# Autodesk Inventor assembly: Hand ASM
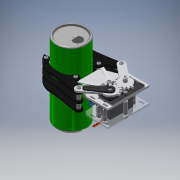
[picture p0: Inventor's stored thumbnail of the model, 180x180]
Saved by Autodesk Inventor 2016 (Build 200138000, 138)
## iProperties
Created: 2017-03-27
Part Number: Hand ASM
Document SubType Name: Assembly
Designer: Nanjar
Author: Nanjar
## Documents named in this file (20)
- D:\Autodesk Invertor prj\Hand Tino Prj2\Hand ASM - Grip.iam
- D:\Autodesk Invertor prj\tower-pro-mg-995-analog-servo-1.snapshot.5\TOWER PRO MG-995, ANALOG SERVO.iam
- D:\Autodesk Invertor prj\Hand Tino Prj\ser Horn.ipt
- D:\Autodesk Invertor prj\Hand Tino Prj\gearb2a.ipt
- D:\Autodesk Invertor prj\Hand Tino Prj\arm1b.ipt
- D:\Autodesk Invertor prj\Hand Tino Prj\claw2.ipt
- D:\Autodesk Invertor prj\Hand Tino Prj\gearb2b.ipt
- D:\Autodesk Invertor prj\arm\spacer 6mm.ipt
- D:\Autodesk Invertor prj\arm\spacer 10mm.ipt
- D:\Autodesk Invertor prj\Gear\Nut90591A121.ipt
- D:\Autodesk Invertor prj\Hand Tino Prj2\Dock bot2.ipt
- D:\Autodesk Invertor prj\Gear\14Screw92005A124.ipt
- D:\Autodesk Invertor prj\Gear\LNut90576A102.ipt
- D:\Autodesk Invertor prj\Gear\10Screw92005A120.ipt
- D:\Autodesk Invertor prj\Gear\20Screw92005A128.ipt
- D:\Autodesk Invertor prj\Hand Tino Prj2\Dock bot1 V2.ipt
- D:\Autodesk Invertor prj\arm\spacer 19mm.ipt
- D:\Autodesk Invertor prj\Downloaded\User Library-HC-SR04\User Library-HC-SR04.iam
- D:\Autodesk Invertor prj\Hand Tino Prj2\Dock top2 V2.ipt
- D:\Autodesk Invertor prj\Hand Tino Prj2\Can1.ipt
## Components (75 placed, 19 different names)
1. TOWER PRO MG-995, ANALOG SERVO:1 [sub-assembly] — Mate:1, Mate:2, Mate:7, Mate:80, Mate:112, Mate:113, Mate:171, Mate:172, Mate:173, Mate:174, Mate:177, Mate:178, Mate:179, Mate:180, Mate:183, Mate:184, Mate:185, Mate:186, Mate:193, Mate:194, Mate:196
2. ser Horn:1 — Mate:1, Mate:2, Mate:6, Mate:8, Mate:81
3. gearb2a:1 — Mate:6, Mate:7, Mate:8, Flush:1, Mate:13, Flush:2, Mate:14, Mate:15, Mate:17, Mate:31, Mate:60, Mate:63, Mate:64, Angle:1, Mate:93, Mate:94, Rotation:1
4. arm1b:1 — Mate:30, Mate:33, Mate:35, Mate:44, Mate:48, Mate:51, Mate:54, Mate:57, Mate:107
5. arm1b:2 — Mate:12, Mate:32, Mate:36, Mate:37, Mate:45, Mate:53, Mate:59, Mate:62, Mate:66
6. claw2:1 — Mate:29, Mate:30, Mate:33, Mate:34, Mate:40, Mate:41, Mate:99, Mate:100, Mate:287, Mate:288, Mate:290
7. claw2:2 — Mate:12, Mate:31, Mate:32, Mate:38, Mate:39, Mate:97, Mate:98, Mate:291, Mate:292, Mate:293, Mate:294
8. gearb2b:1 — Flush:1, Mate:16, Mate:17, Mate:29, Mate:47, Mate:50, Mate:56, Mate:69, Mate:72, Mate:79, Mate:95, Mate:96, Rotation:1
9. spacer 10mm:2 — Mate:34, Mate:35, Mate:49
10. spacer 10mm:3 — Mate:36, Mate:37, Mate:61
11. spacer 10mm:4 — Mate:38, Mate:39
12. spacer 10mm:5 — Mate:40, Mate:41
13. Dock bot2:1 — Mate:44, Mate:45, Mate:51, Mate:53, Mate:107, Mate:110, Mate:111, Mate:299, Mate:300, Mate:301
14. claw2:3 — Mate:47, Mate:48, Mate:49, Mate:52, Mate:55, Mate:313
15. spacer 10mm:7 — Mate:54, Mate:55, Mate:58, Mate:267
16. spacer 10mm:8 — Mate:50, Mate:52, Mate:266
17. claw2:4 — Mate:56, Mate:57, Mate:58, Mate:262, Mate:264, Mate:316
18. claw2:5 — Mate:59, Mate:60, Mate:61, Mate:65, Mate:67, Mate:311
19. claw2:6 — Mate:62, Mate:63, Mate:68, Mate:263, Mate:265, Mate:314
20. spacer 10mm:9 — Mate:64, Mate:65, Mate:268
21. spacer 10mm:10 — Mate:66, Mate:67, Mate:68, Mate:269
22. 14Screw92005A124:1 — Mate:72, Mate:77, Mate:309
23. Nut90591A121:2 — Mate:69, Mate:78, Mate:79
24. LNut90576A102:1 — Mate:77, Mate:78
25. 10Screw92005A120:1 — Mate:80, Mate:81
26. Nut90591A121:3
27. 10Screw92005A120:5 — Mate:93, Mate:94
28. 10Screw92005A120:7 — Mate:95, Mate:96
29. 10Screw92005A120:8 — Mate:97, Mate:98
30. 10Screw92005A120:9 — Mate:99, Mate:100
31. 20Screw92005A128:1 — Mate:283, Mate:305, Mate:308
32. 20Screw92005A128:2 — Mate:110
33. 20Screw92005A128:3 — Mate:111, Mate:270
34. Dock bot1 V2:1 — Mate:112, Mate:113, Mate:189, Mate:190, Mate:191, Mate:192, Mate:197, Mate:198, Mate:199, Mate:200, Mate:271, Mate:272, Mate:273, Mate:274, Mate:276, Mate:278, Mate:280, Mate:282, Mate:284, Mate:286
35. 20Screw92005A128:4 — Mate:275, Mate:306, Mate:307
36. spacer 6mm:9 — Mate:169, Mate:170
37. spacer 10mm:13 — Mate:169, Mate:170, Mate:171, Mate:172
38. Nut90591A121:7 — Mate:173, Mate:174
39. spacer 6mm:10
40. spacer 10mm:14 — Mate:179, Mate:180
41. Nut90591A121:8 — Mate:177, Mate:178
42. spacer 6mm:11
43. spacer 10mm:15 — Mate:183, Mate:184
44. Nut90591A121:9 — Mate:185, Mate:186
45. spacer 6mm:12
46. spacer 10mm:16 — Mate:193, Mate:194, Mate:195
47. Nut90591A121:10 — Mate:195, Mate:196
48. 10Screw92005A120:10 — Mate:189, Mate:190
49. 10Screw92005A120:11 — Mate:191, Mate:192
50. 10Screw92005A120:12 — Mate:197, Mate:200
51. 10Screw92005A120:13 — Mate:198, Mate:199
52. Nut90591A121:16 — Mate:262, Mate:266
53. Nut90591A121:17 — Mate:263, Mate:268
54. Nut90591A121:18 — Mate:264, Mate:267
55. Nut90591A121:19 — Mate:265, Mate:269
56. spacer 19mm:1 — Mate:270, Mate:271, Mate:272, Mate:279
57. spacer 19mm:2 — Mate:273, Mate:274, Mate:277
58. spacer 19mm:3 — Mate:275, Mate:276, Mate:281
59. Nut90591A121:20 — Mate:277, Mate:278
60. Nut90591A121:21 — Mate:279, Mate:280
61. Nut90591A121:22 — Mate:281, Mate:282
62. spacer 19mm:4 — Mate:283, Mate:284, Mate:285
63. Nut90591A121:23 — Mate:285, Mate:286
64. User Library-HC-SR04:2 [sub-assembly]
65. spacer 10mm:17 — Mate:287, Mate:288, Mate:289, Mate:312
66. 10Screw92005A120:19 — Mate:289, Mate:290
67. spacer 10mm:18 — Mate:291, Mate:292, Mate:310
68. 10Screw92005A120:20 — Mate:293, Mate:294
69. Dock top2 V2:1 — Mate:299, Mate:300, Mate:301, Mate:302, Mate:303, Mate:304
70. Dock top2 V2:2 — Mate:302, Mate:303, Mate:304, Mate:305, Mate:306, Mate:307, Mate:308, Mate:309
71. spacer 10mm:19 — Mate:310, Mate:311, Mate:315
72. spacer 10mm:20 — Mate:312, Mate:313, Mate:317
73. Nut90591A121:24 — Mate:314, Mate:315
74. Nut90591A121:25 — Mate:316, Mate:317
75. Can1:1 — Flush:3
## Relationships (157: Mate 152, Flush 3, Angle 1, RelateRotation 1)
- Mate:1: TOWER PRO MG-995, ANALOG SERVO:1 ↔ ser Horn:1
- Mate:2: TOWER PRO MG-995, ANALOG SERVO:1 ↔ ser Horn:1
- Mate:6: ser Horn:1 ↔ gearb2a:1
- Mate:7: TOWER PRO MG-995, ANALOG SERVO:1 ↔ gearb2a:1
- Mate:8: ser Horn:1 ↔ gearb2a:1
- Mate:12: arm1b:2 ↔ claw2:2
- Flush:1: gearb2a:1 ↔ gearb2b:1
- Mate:13: gearb2a:1
- Flush:2: gearb2a:1
- Mate:14: gearb2a:1
- Mate:15: gearb2a:1
- Mate:16: gearb2b:1
- Mate:17 (26.23 mm): gearb2a:1 ↔ gearb2b:1
- Mate:29: claw2:1 ↔ gearb2b:1
- Mate:30: arm1b:1 ↔ claw2:1
- Mate:31: gearb2a:1 ↔ claw2:2
- Mate:32: arm1b:2 ↔ claw2:2
- Mate:33: arm1b:1 ↔ claw2:1
- Mate:34: claw2:1 ↔ spacer 10mm:2
- Mate:35: arm1b:1 ↔ spacer 10mm:2
- Mate:36: arm1b:2 ↔ spacer 10mm:3
- Mate:37: arm1b:2 ↔ spacer 10mm:3
- Mate:38: claw2:2 ↔ spacer 10mm:4
- Mate:39: claw2:2 ↔ spacer 10mm:4
- Mate:40: claw2:1 ↔ spacer 10mm:5
- Mate:41: claw2:1 ↔ spacer 10mm:5
- Mate:44: arm1b:1 ↔ Dock bot2:1
- Mate:45: arm1b:2 ↔ Dock bot2:1
- Mate:47: gearb2b:1 ↔ claw2:3
- Mate:48: arm1b:1 ↔ claw2:3
- Mate:49: spacer 10mm:2 ↔ claw2:3
- Mate:50: gearb2b:1 ↔ spacer 10mm:8
- Mate:51: arm1b:1 ↔ Dock bot2:1
- Mate:52: claw2:3 ↔ spacer 10mm:8
- Mate:53: arm1b:2 ↔ Dock bot2:1
- Mate:54: arm1b:1 ↔ spacer 10mm:7
- Mate:55: claw2:3 ↔ spacer 10mm:7
- Mate:56: gearb2b:1 ↔ claw2:4
- Mate:57: arm1b:1 ↔ claw2:4
- Mate:58: spacer 10mm:7 ↔ claw2:4
- Mate:59: arm1b:2 ↔ claw2:5
- Mate:60: gearb2a:1 ↔ claw2:5
- Mate:61: spacer 10mm:3 ↔ claw2:5
- Mate:62: arm1b:2 ↔ claw2:6
- Mate:63: gearb2a:1 ↔ claw2:6
- Mate:64: gearb2a:1 ↔ spacer 10mm:9
- Mate:65: claw2:5 ↔ spacer 10mm:9
- Mate:66: arm1b:2 ↔ spacer 10mm:10
- Mate:67: claw2:5 ↔ spacer 10mm:10
- Mate:68: claw2:6 ↔ spacer 10mm:10
- Angle:1 (142 deg): gearb2a:1
- Mate:69: gearb2b:1 ↔ Nut90591A121:2
- Mate:72: gearb2b:1 ↔ 14Screw92005A124:1
- Mate:77: 14Screw92005A124:1 ↔ LNut90576A102:1
- Mate:78: Nut90591A121:2 ↔ LNut90576A102:1
- Mate:79: gearb2b:1 ↔ Nut90591A121:2
- Mate:80: TOWER PRO MG-995, ANALOG SERVO:1 ↔ 10Screw92005A120:1
- Mate:81: ser Horn:1 ↔ 10Screw92005A120:1
- Mate:93: gearb2a:1 ↔ 10Screw92005A120:5
- Mate:94: gearb2a:1 ↔ 10Screw92005A120:5
- Mate:95: gearb2b:1 ↔ 10Screw92005A120:7
- Mate:96: gearb2b:1 ↔ 10Screw92005A120:7
- Mate:97: claw2:2 ↔ 10Screw92005A120:8
- Mate:98: claw2:2 ↔ 10Screw92005A120:8
- Mate:99: claw2:1 ↔ 10Screw92005A120:9
- Mate:100: claw2:1 ↔ 10Screw92005A120:9
- Mate:107: arm1b:1 ↔ Dock bot2:1
- Mate:110: Dock bot2:1 ↔ 20Screw92005A128:2
- Mate:111: Dock bot2:1 ↔ 20Screw92005A128:3
- Mate:112: TOWER PRO MG-995, ANALOG SERVO:1 ↔ Dock bot1 V2:1
- Mate:113: TOWER PRO MG-995, ANALOG SERVO:1 ↔ Dock bot1 V2:1
- Mate:169: spacer 6mm:9 ↔ spacer 10mm:13
- Mate:170 (0.4 mm): spacer 6mm:9 ↔ spacer 10mm:13
- Mate:171: TOWER PRO MG-995, ANALOG SERVO:1 ↔ spacer 10mm:13
- Mate:172: TOWER PRO MG-995, ANALOG SERVO:1 ↔ spacer 10mm:13
- Mate:173: TOWER PRO MG-995, ANALOG SERVO:1 ↔ Nut90591A121:7
- Mate:174: TOWER PRO MG-995, ANALOG SERVO:1 ↔ Nut90591A121:7
- [Mate]: spacer 6mm:10 ↔ spacer 10mm:14
- [Mate] (0.4 mm): spacer 6mm:10 ↔ spacer 10mm:14
- Mate:177: TOWER PRO MG-995, ANALOG SERVO:1 ↔ Nut90591A121:8
- Mate:178: TOWER PRO MG-995, ANALOG SERVO:1 ↔ Nut90591A121:8
- Mate:179: TOWER PRO MG-995, ANALOG SERVO:1 ↔ spacer 10mm:14
- Mate:180: TOWER PRO MG-995, ANALOG SERVO:1 ↔ spacer 10mm:14
- [Mate]: spacer 6mm:11 ↔ spacer 10mm:15
- [Mate] (0.4 mm): spacer 6mm:11 ↔ spacer 10mm:15
- Mate:183: TOWER PRO MG-995, ANALOG SERVO:1 ↔ spacer 10mm:15
- Mate:184: TOWER PRO MG-995, ANALOG SERVO:1 ↔ spacer 10mm:15
- Mate:185: TOWER PRO MG-995, ANALOG SERVO:1 ↔ Nut90591A121:9
- Mate:186: TOWER PRO MG-995, ANALOG SERVO:1 ↔ Nut90591A121:9
- [Mate]: spacer 6mm:12 ↔ spacer 10mm:16
- [Mate] (0.4 mm): spacer 6mm:12 ↔ spacer 10mm:16
- Mate:189: Dock bot1 V2:1 ↔ 10Screw92005A120:10
- Mate:190: Dock bot1 V2:1 ↔ 10Screw92005A120:10
- Mate:191: Dock bot1 V2:1 ↔ 10Screw92005A120:11
- Mate:192: Dock bot1 V2:1 ↔ 10Screw92005A120:11
- Mate:193: TOWER PRO MG-995, ANALOG SERVO:1 ↔ spacer 10mm:16
- Mate:194: TOWER PRO MG-995, ANALOG SERVO:1 ↔ spacer 10mm:16
- Mate:195: spacer 10mm:16 ↔ Nut90591A121:10
- Mate:196: TOWER PRO MG-995, ANALOG SERVO:1 ↔ Nut90591A121:10
- Mate:197: Dock bot1 V2:1 ↔ 10Screw92005A120:12
- Mate:198: Dock bot1 V2:1 ↔ 10Screw92005A120:13
- Mate:199: Dock bot1 V2:1 ↔ 10Screw92005A120:13
- Mate:200: Dock bot1 V2:1 ↔ 10Screw92005A120:12
- Mate:262: claw2:4 ↔ Nut90591A121:16
- Mate:263: claw2:6 ↔ Nut90591A121:17
- Mate:264: claw2:4 ↔ Nut90591A121:18
- Mate:265: claw2:6 ↔ Nut90591A121:19
- Mate:266: spacer 10mm:8 ↔ Nut90591A121:16
- Mate:267: spacer 10mm:7 ↔ Nut90591A121:18
- Mate:268: spacer 10mm:9 ↔ Nut90591A121:17
- Mate:269: spacer 10mm:10 ↔ Nut90591A121:19
- Mate:270: 20Screw92005A128:3 ↔ spacer 19mm:1
- Mate:271: Dock bot1 V2:1 ↔ spacer 19mm:1
- Mate:272: Dock bot1 V2:1 ↔ spacer 19mm:1
- Mate:273: Dock bot1 V2:1 ↔ spacer 19mm:2
- Mate:274: Dock bot1 V2:1 ↔ spacer 19mm:2
- Mate:275: 20Screw92005A128:4 ↔ spacer 19mm:3
- Mate:276: Dock bot1 V2:1 ↔ spacer 19mm:3
- Mate:277: spacer 19mm:2 ↔ Nut90591A121:20
- Mate:278: Dock bot1 V2:1 ↔ Nut90591A121:20
- Mate:279: spacer 19mm:1 ↔ Nut90591A121:21
- Mate:280: Dock bot1 V2:1 ↔ Nut90591A121:21
- Mate:281: spacer 19mm:3 ↔ Nut90591A121:22
- Mate:282: Dock bot1 V2:1 ↔ Nut90591A121:22
- Mate:283: 20Screw92005A128:1 ↔ spacer 19mm:4
- Mate:284: Dock bot1 V2:1 ↔ spacer 19mm:4
- Mate:285: spacer 19mm:4 ↔ Nut90591A121:23
- Mate:286: Dock bot1 V2:1 ↔ Nut90591A121:23
- Mate:287: claw2:1 ↔ spacer 10mm:17
- Mate:288: claw2:1 ↔ spacer 10mm:17
- Mate:289: spacer 10mm:17 ↔ 10Screw92005A120:19
- Mate:290: claw2:1 ↔ 10Screw92005A120:19
- Mate:291: claw2:2 ↔ spacer 10mm:18
- Mate:292: claw2:2 ↔ spacer 10mm:18
- Mate:293: claw2:2 ↔ 10Screw92005A120:20
- Mate:294: claw2:2 ↔ 10Screw92005A120:20
- Mate:299: Dock bot2:1 ↔ Dock top2 V2:1
- Mate:300: Dock bot2:1 ↔ Dock top2 V2:1
- Mate:301: Dock bot2:1 ↔ Dock top2 V2:1
- Mate:302: Dock top2 V2:1 ↔ Dock top2 V2:2
- Mate:303: Dock top2 V2:1 ↔ Dock top2 V2:2
- Mate:304: Dock top2 V2:1 ↔ Dock top2 V2:2
- Mate:305: 20Screw92005A128:1 ↔ Dock top2 V2:2
- Mate:306: 20Screw92005A128:4 ↔ Dock top2 V2:2
- Mate:307: 20Screw92005A128:4 ↔ Dock top2 V2:2
- Mate:308: 20Screw92005A128:1 ↔ Dock top2 V2:2
- Mate:309: 14Screw92005A124:1 ↔ Dock top2 V2:2
- Mate:310: spacer 10mm:18 ↔ spacer 10mm:19
- Mate:311: claw2:5 ↔ spacer 10mm:19
- Mate:312: spacer 10mm:17 ↔ spacer 10mm:20
- Mate:313: claw2:3 ↔ spacer 10mm:20
- Mate:314: claw2:6 ↔ Nut90591A121:24
- Mate:315: spacer 10mm:19 ↔ Nut90591A121:24
- Mate:316: claw2:4 ↔ Nut90591A121:25
- Mate:317: spacer 10mm:20 ↔ Nut90591A121:25
- Rotation:1 [RelateRotation] (1 ul): gearb2a:1 ↔ gearb2b:1
- Flush:3 (-35 mm): Can1:1
## Named parameters: d224_d218 = 0 mm, d225_d219 = 0.4 mm, d230_d218 = 0 mm, d231_d219 = 0.4 mm, d236_d218 = 0 mm, d237_d219 = 0.4 mm
